# Autodesk Inventor assembly: Zusammenbau_Mehrmodul
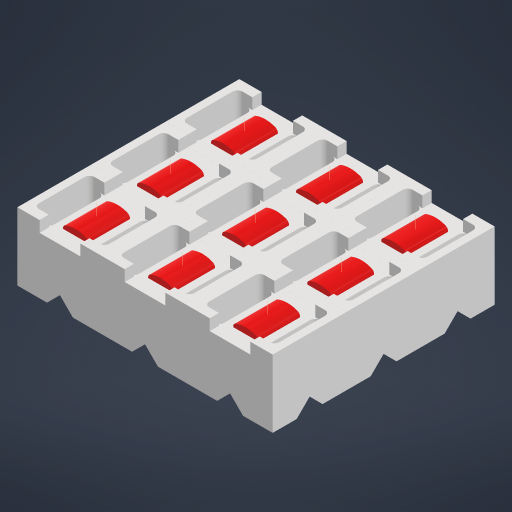
[picture p0: Inventor's stored thumbnail of the model, 512x512]
Saved by Autodesk Inventor 2023 (Build 270158030, 158C)
## iProperties
Created: 2022-05-12
Part Number: Zusammenbau_Mehrmodul
Document SubType Name: Assembly
Designer: Simon
Author: Simon
## Documents named in this file (2)
- C:\Users\simfe\Desktop\2.Semester\Technische Grundlagen-II\Pixie\3d-modelle\.iam's\Zusammenbau_Mehrmodul.iam
- C:\Users\simfe\Desktop\2.Semester\Technische Grundlagen-II\Pixie\3d-modelle\.iam's\Zusammenbau_Einzelmodul.iam
## Components (9 placed, 1 different names)
1. Zusammenbau_Einzelmodul:1 [sub-assembly] — Mate:1, Flush:1, Flush:2, Mate:2, Flush:3, Flush:4
2. Zusammenbau_Einzelmodul:2 [sub-assembly] — Mate:1, Flush:1, Flush:2, Mate:4, Mate:5, Flush:6, Flush:7
3. Zusammenbau_Einzelmodul:3 [sub-assembly] — Mate:2, Flush:3, Flush:4, Mate:3, Flush:5, Mate:8, Flush:9, Flush:10
4. Zusammenbau_Einzelmodul:4 [sub-assembly] — Mate:3, Mate:4, Flush:5, Mate:7, Flush:8
5. Zusammenbau_Einzelmodul:5 [sub-assembly] — Mate:6, Mate:7, Flush:8, Flush:13
6. Zusammenbau_Einzelmodul:6 [sub-assembly] — Mate:5, Flush:6, Flush:7, Mate:6
7. Zusammenbau_Einzelmodul:7 [sub-assembly] — Mate:8, Flush:9, Flush:10, Flush:11, Flush:12, Mate:9
8. Zusammenbau_Einzelmodul:8 [sub-assembly] — Flush:11, Flush:12, Mate:9, Flush:14, Flush:15
9. Zusammenbau_Einzelmodul:9 [sub-assembly] — Flush:13, Flush:14, Flush:15
## Relationships (24: Flush 15, Mate 9)
- Mate:1: Zusammenbau_Einzelmodul:1 ↔ Zusammenbau_Einzelmodul:2
- Flush:1: Zusammenbau_Einzelmodul:1 ↔ Zusammenbau_Einzelmodul:2
- Flush:2: Zusammenbau_Einzelmodul:1 ↔ Zusammenbau_Einzelmodul:2
- Mate:2: Zusammenbau_Einzelmodul:1 ↔ Zusammenbau_Einzelmodul:3
- Flush:3: Zusammenbau_Einzelmodul:1 ↔ Zusammenbau_Einzelmodul:3
- Flush:4: Zusammenbau_Einzelmodul:1 ↔ Zusammenbau_Einzelmodul:3
- Mate:3: Zusammenbau_Einzelmodul:3 ↔ Zusammenbau_Einzelmodul:4
- Mate:4: Zusammenbau_Einzelmodul:2 ↔ Zusammenbau_Einzelmodul:4
- Flush:5: Zusammenbau_Einzelmodul:3 ↔ Zusammenbau_Einzelmodul:4
- Mate:5: Zusammenbau_Einzelmodul:2 ↔ Zusammenbau_Einzelmodul:6
- Flush:6: Zusammenbau_Einzelmodul:2 ↔ Zusammenbau_Einzelmodul:6
- Flush:7: Zusammenbau_Einzelmodul:2 ↔ Zusammenbau_Einzelmodul:6
- Mate:6: Zusammenbau_Einzelmodul:5 ↔ Zusammenbau_Einzelmodul:6
- Mate:7: Zusammenbau_Einzelmodul:4 ↔ Zusammenbau_Einzelmodul:5
- Flush:8: Zusammenbau_Einzelmodul:4 ↔ Zusammenbau_Einzelmodul:5
- Mate:8: Zusammenbau_Einzelmodul:3 ↔ Zusammenbau_Einzelmodul:7
- Flush:9: Zusammenbau_Einzelmodul:3 ↔ Zusammenbau_Einzelmodul:7
- Flush:10: Zusammenbau_Einzelmodul:3 ↔ Zusammenbau_Einzelmodul:7
- Flush:11: Zusammenbau_Einzelmodul:7 ↔ Zusammenbau_Einzelmodul:8
- Flush:12: Zusammenbau_Einzelmodul:7 ↔ Zusammenbau_Einzelmodul:8
- Mate:9: Zusammenbau_Einzelmodul:7 ↔ Zusammenbau_Einzelmodul:8
- Flush:13: Zusammenbau_Einzelmodul:5 ↔ Zusammenbau_Einzelmodul:9
- Flush:14: Zusammenbau_Einzelmodul:8 ↔ Zusammenbau_Einzelmodul:9
- Flush:15: Zusammenbau_Einzelmodul:8 ↔ Zusammenbau_Einzelmodul:9
